# Autodesk Inventor assembly: Assembly31
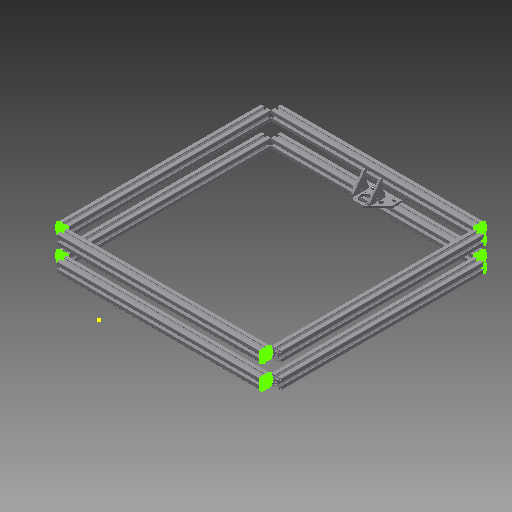
[picture p0: Inventor's stored thumbnail of the model, 512x512]
Saved by Autodesk Inventor 2017 (Build 210142000, 142)
## iProperties
Created: 2016-08-03
Part Number: Assembly31
Document SubType Name: Assembly
Designer: User
Author: User
## Documents named in this file (3)
- C:\All INVENTOR\SL-Inventor\SL-Beast 3D Printer\Assembly31.iam
- C:\All INVENTOR\SL-Inventor\SL-Beast 3D Printer\3030 600mm.ipt
- C:\All INVENTOR\SL-Inventor\SL-Beast 3D Printer\RearZMotorMount.iam
## Components (7 placed, 2 different names)
1. 3030 600mm:1
2. 3030 600mm:2
3. 3030 600mm:3
4. 3030 600mm:4
5. 3030 600mm:5
6. 3030 600mm:6
7. RearZMotorMount:1 [sub-assembly]
## Relationships (5: Flush 4, Mate 1)
- [Flush]: 3030 600mm:2 ↔ 3030 600mm:4
- [Flush]: 3030 600mm:2 ↔ 3030 600mm:5
- [Flush]: 3030 600mm:3 ↔ RearZMotorMount:1
- [Flush]: 3030 600mm:4 ↔ RearZMotorMount:1
- [Mate]: 3030 600mm:2 ↔ RearZMotorMount:1
